# Autodesk Inventor assembly: Turret_Assem
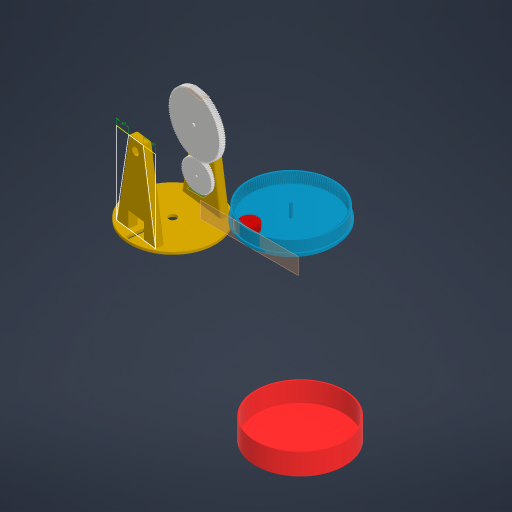
[picture p0: Inventor's stored thumbnail of the model, 512x512]
Saved by Autodesk Inventor 2023 (Build 270158000, 158)
## iProperties
Created: 2022-05-13
Part Number: Turret_Assem
Document SubType Name: Assembly
Designer: jayso
Author: jayso
## Documents named in this file (7)
- C:\Users\jayso\Desktop\Turret_CAD\CAD\Turret_Assem.iam
- C:\Users\jayso\Desktop\Turret_CAD\CAD\electronics-base.ipt
- C:\Users\jayso\Desktop\Turret_CAD\CAD\electronics-cover.ipt
- C:\Users\jayso\Desktop\Turret_CAD\CAD\y-axis-gear.ipt
- C:\Users\jayso\Desktop\Turret_CAD\CAD\x-axis-gear.ipt
- C:\Users\jayso\Desktop\Turret_CAD\CAD\turret-base.ipt
- C:\Users\jayso\Desktop\Turret_CAD\CAD\shooter-right-shaft-attach.ipt
## Components (6 placed, 6 different names)
1. electronics-base:1
2. electronics-cover:1 — Mate:1
3. y-axis-gear:1 — Mate:1
4. x-axis-gear:1
5. turret-base:1 — Rigid:1
6. shooter-right-shaft-attach:1 — Rigid:1
## Relationships (2: WeldJoint 1, Mate 1)
- Rigid:1 [WeldJoint] (20.6375 mm): turret-base:1 ↔ shooter-right-shaft-attach:1
- Mate:1: electronics-cover:1 ↔ y-axis-gear:1
